# Autodesk Inventor assembly: 22-134
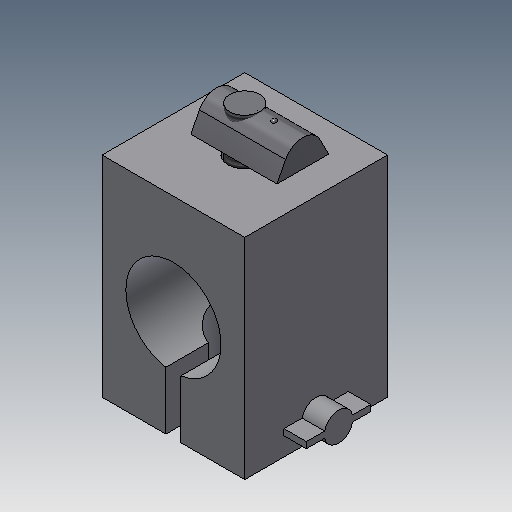
[picture p0: Inventor's stored thumbnail of the model, 512x512]
Saved by Autodesk Inventor 2018.3 (Build 223284000, 284)
## iProperties
Created: 2004-11-24
Part Number: 22-134
Document SubType Name: Assembly
Designer: Autodesk, Inc.
Manufacturer: Standard
Standards Organization: Custom
Description: SLIDE COLLAR
Vendor: PARKER IPS
Catalog Web Link: http://www.parker.com/ead/cm1.asp?cmid=809
Mass: 78.0709 g
Surface Area: 169.539 cm^2
Volume: 58.5245 cm^3
Density: 1.33399 g/cm^3
CAGE: 1LJX3
Dept. ID: Product Design
Description #2: ---
Finish #1: ---
Finish #2: ---
Material ID: ---
Project Number: ---
Author: Autodesk, Inc.
## Documents named in this file (6)
- C:\AVAInvAPI\Workspace\Test Station\Components\22-134.iam
- C:\AVAInvAPI\Workspace\Test Station\Components\24-120-8.ipt
- C:\AVAInvAPI\Workspace\Test Station\Components\20-058.ipt
- C:\AVAInvAPI\Workspace\Test Station\Components\22-134.ipt
- C:\Users\kelleyb.ADS\Desktop\Samples MIGRATED 2009 224 RTM_1\Standard Parts\Test Station Content\Fastners\2X-YYY-ZZ IPS Screws.ipt
- C:\Users\kelleyb.ADS\Desktop\Samples MIGRATED 2009 224 RTM_1\Standard Parts\Test Station Content\Fastners\20-XXX TSlot Nuts.ipt
## Components (3 placed, 3 different names)
1. 22-134:1 — Insert:1, Mate:1, Angle:1
2. 24-120-8:1 — Insert:1, Mate:2
3. 20-058:1 — Mate:1, Mate:2, Angle:1
## Relationships (4: Mate 2, Insert 1, Angle 1)
- Insert:1: 22-134:1 ↔ 24-120-8:1
- Mate:1 (4.5 mm): 22-134:1 ↔ 20-058:1
- Mate:2: 24-120-8:1 ↔ 20-058:1
- Angle:1 (0 deg): 22-134:1 ↔ 20-058:1
